# Autodesk Inventor assembly: DriveTrainAssembly
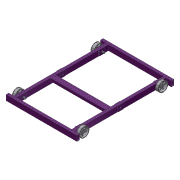
[picture p0: Inventor's stored thumbnail of the model, 180x180]
Saved by Autodesk Inventor 2012 (Build 160160000, 160)
## iProperties
Created: 2012-11-20
Part Number: DriveTrainAssembly
Document SubType Name: Assembly
Designer: JesseK
Author: JesseK
## Documents named in this file (4)
- Z:\UserData\Documents\Inventor\team1885frc\Robot2013\DriveTrainProto\DriveTrainAssembly.iam
- Z:\UserData\Documents\Inventor\team1885frc\Robot2013\DriveTrainProto\DriveTrainFrame.iam
- Z:\UserData\Documents\Inventor\team1885frc\Robot2013\DriveTrainProto\OuterAxle.ipt
- Z:\UserData\Documents\Inventor\team1885frc\AndyMark\4+Performance+Keyed+2.ipt
## Components (9 placed, 3 different names)
1. DriveTrainFrame:1 [sub-assembly] — Mate:1, Flush:1, Flush:2, Mate:2, Flush:3, Mate:3, Flush:4, Mate:4, Mate:5, Mate:7, Mate:9, Mate:11
2. OuterAxle:1 — Mate:1, Flush:1, Mate:10
3. OuterAxle:2 — Flush:2, Mate:2, Mate:12
4. OuterAxle:3 — Flush:3, Mate:3, Mate:8
5. OuterAxle:4 — Flush:4, Mate:4, Mate:6
6. 4+Performance+Keyed+2:1 — Mate:5, Mate:6
7. 4+Performance+Keyed+2:2 — Mate:9, Mate:10
8. 4+Performance+Keyed+2:3 — Mate:7, Mate:8
9. 4+Performance+Keyed+2:4 — Mate:11, Mate:12
## Relationships (16: Mate 12, Flush 4)
- Mate:1: DriveTrainFrame:1 ↔ OuterAxle:1
- Flush:1: DriveTrainFrame:1 ↔ OuterAxle:1
- Flush:2: DriveTrainFrame:1 ↔ OuterAxle:2
- Mate:2: DriveTrainFrame:1 ↔ OuterAxle:2
- Flush:3: DriveTrainFrame:1 ↔ OuterAxle:3
- Mate:3: DriveTrainFrame:1 ↔ OuterAxle:3
- Flush:4: DriveTrainFrame:1 ↔ OuterAxle:4
- Mate:4: DriveTrainFrame:1 ↔ OuterAxle:4
- Mate:5 (1.5875 mm): DriveTrainFrame:1 ↔ 4+Performance+Keyed+2:1
- Mate:6: OuterAxle:4 ↔ 4+Performance+Keyed+2:1
- Mate:7 (1.5875 mm): DriveTrainFrame:1 ↔ 4+Performance+Keyed+2:3
- Mate:8: OuterAxle:3 ↔ 4+Performance+Keyed+2:3
- Mate:9 (1.5875 mm): DriveTrainFrame:1 ↔ 4+Performance+Keyed+2:2
- Mate:10: OuterAxle:1 ↔ 4+Performance+Keyed+2:2
- Mate:11 (1.5875 mm): DriveTrainFrame:1 ↔ 4+Performance+Keyed+2:4
- Mate:12: OuterAxle:2 ↔ 4+Performance+Keyed+2:4
